# Autodesk Inventor assembly: arm j4 assembly
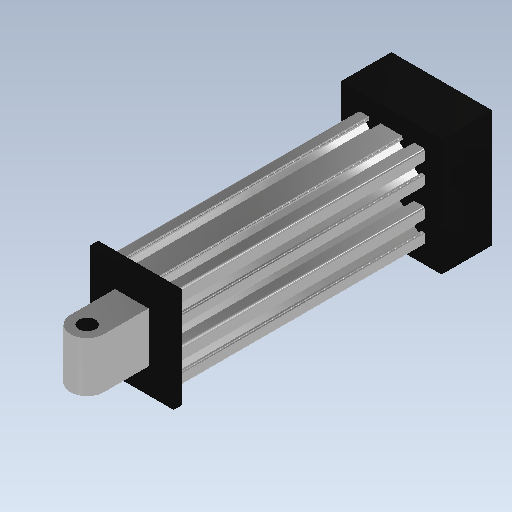
[picture p0: Inventor's stored thumbnail of the model, 512x512]
Saved by Autodesk Inventor 2020 (Build 240168000, 168)
## iProperties
Created: 2020-07-11
Part Number: arm j4 assembly
Document SubType Name: Assembly
Designer: Vikki
Mass: 243.922 g
Surface Area: 1219.05 cm^2
Volume: 243.922 cm^3
Density: 1 g/cm^3
Author: Vikki
## Documents named in this file (3)
- E:\project inventor pro\flipkart grid models\articulated arm\arm j4 assembly.iam
- E:\project inventor pro\flipkart grid models\articulated arm\j4 for end effector.ipt
- E:\project inventor pro\flipkart grid models\articulated arm\alm ext 2040 150mm.ipt
## Components (2 placed, 2 different names)
1. j4 for end effector:1 — Mate:1, Mate:2, Flush:1, Flush:2
2. alm ext 2040 150mm:1 — Mate:1, Mate:2, Flush:1, Flush:2
## Relationships (4: Mate 2, Flush 2)
- Mate:1: j4 for end effector:1 ↔ alm ext 2040 150mm:1
- Mate:2: j4 for end effector:1 ↔ alm ext 2040 150mm:1
- Flush:1: j4 for end effector:1 ↔ alm ext 2040 150mm:1
- Flush:2: j4 for end effector:1 ↔ alm ext 2040 150mm:1
